# Autodesk Inventor assembly: ensamble engranes Fernando Meneses 1052621
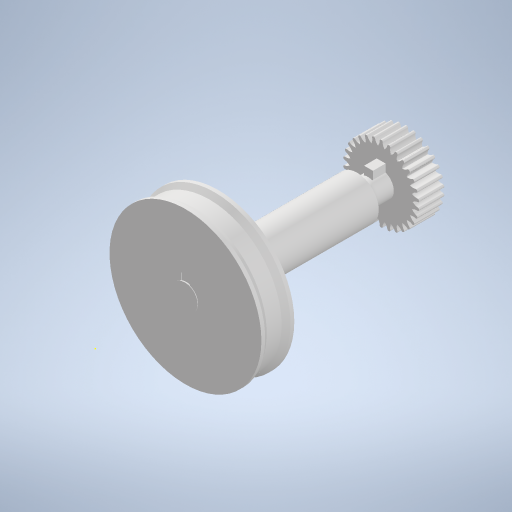
[picture p0: Inventor's stored thumbnail of the model, 512x512]
Saved by Autodesk Inventor 2024 (Build 280153000, 153)
## iProperties
Created: 2024-03-31
Part Number: ensamble engranes Fernando Meneses 1052621
Document SubType Name: Assembly
Designer: menes
Author: menes
## Documents named in this file (6)
- C:\Users\menes\OneDrive\Documentos\Primer ciclo 2024\Dinamica lab\ensamble engranes Fernando Meneses 1052621.iam
- C:\Users\menes\OneDrive\Documentos\Primer ciclo 2024\Dinamica lab\CUÑA.ipt
- C:\Users\menes\OneDrive\Documentos\Primer ciclo 2024\Dinamica lab\EJE_CUÑEROS.ipt
- C:\Users\menes\OneDrive\Documentos\Primer ciclo 2024\Dinamica lab\ENGRANE.ipt
- C:\Users\menes\OneDrive\Documentos\Primer ciclo 2024\Dinamica lab\POLEA.ipt
- C:\Users\menes\OneDrive\Documentos\Primer ciclo 2024\Dinamica lab\parte adicional.ipt
## Components (7 placed, 5 different names)
1. CUÑA:1 — Mate:2
2. EJE_CUÑEROS:1 — Mate:1, Mate:2, Mate:3, Mate:4, Mate:5, Mate:6
3. ENGRANE:1 — Mate:4
4. POLEA:1 — Mate:1
5. CUÑA:2 — Mate:3
6. CUÑA:3 — Mate:5
7. parte adicional:1 — Mate:6
## Relationships (6: Mate 6)
- Mate:1: EJE_CUÑEROS:1 ↔ POLEA:1
- Mate:2: CUÑA:1 ↔ EJE_CUÑEROS:1
- Mate:3: EJE_CUÑEROS:1 ↔ CUÑA:2
- Mate:4: EJE_CUÑEROS:1 ↔ ENGRANE:1
- Mate:5: EJE_CUÑEROS:1 ↔ CUÑA:3
- Mate:6: EJE_CUÑEROS:1 ↔ parte adicional:1
